# Autodesk Inventor assembly: mech_wheel_assembly
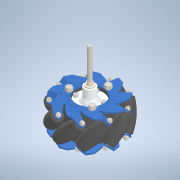
[picture p0: Inventor's stored thumbnail of the model, 180x180]
Saved by Autodesk Inventor 2020 (Build 240168000, 168)
## iProperties
Created: 2019-09-11
Part Number: mech_wheel_assembly
Document SubType Name: Assembly
Designer: tbloo
Author: tbloo
## Documents named in this file (4)
- D:\Documents\GitHub\AO_Robotics\CAD\Projects\Timothy Bloot\mech_wheel_assembly.iam
- D:\Documents\GitHub\AO_Robotics\CAD\Parts Kits\FTC Tetrix KOP Organized (7-24-19)\Wheel\Mechanum Wheel\left_a_mecanum wheel.ipt
- D:\Documents\GitHub\AO_Robotics\CAD\Parts Kits\FTC Tetrix KOP Organized (7-24-19)\Axle Hardware\Tetrix_40225-80mm.ipt
- D:\Documents\GitHub\AO_Robotics\CAD\Parts Kits\FTC Tetrix KOP Organized (7-24-19)\Axle Hardware\AM_6mm_Bushing.ipt
## Components (4 placed, 3 different names)
1. left_a_mecanum wheel:1 — Rotational:1, Rotational:2
2. Tetrix_40225-80mm:1 — Rotational:2, Rotational:3
3. AM_6mm_Bushing:1 — Rotational:1
4. AM_6mm_Bushing:2 — Rotational:3
## Relationships (3: RevoluteJoint 3)
- Rotational:1 [RevoluteJoint]: left_a_mecanum wheel:1 ↔ AM_6mm_Bushing:1
- Rotational:2 [RevoluteJoint]: left_a_mecanum wheel:1 ↔ Tetrix_40225-80mm:1
- Rotational:3 [RevoluteJoint] (-18.3 mm): Tetrix_40225-80mm:1 ↔ AM_6mm_Bushing:2
